# Autodesk Inventor assembly: gameMech_pegged
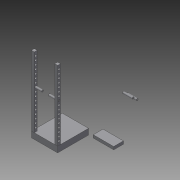
[picture p0: Inventor's stored thumbnail of the model, 180x180]
Saved by Autodesk Inventor 2015 (Build 190159000, 159)
## iProperties
Created: 2015-01-15
Part Number: gameMech_pegged
Document SubType Name: Assembly
Designer: Tucker
Author: Tucker
## Documents named in this file (5)
- C:\Users\Tucker\Documents\GitHub\frc2015\CAD\gameMech_pegged.iam
- C:\Users\Tucker\Documents\GitHub\frc2015\CAD\chasse.ipt
- C:\Users\Tucker\Documents\GitHub\frc2015\CAD\pole.ipt
- C:\Users\Tucker\Documents\GitHub\frc2015\CAD\box_forklift.ipt
- C:\Users\Tucker\Documents\GitHub\frc2015\CAD\axle_word_used_loosely.ipt
## Components (8 placed, 4 different names)
1. chasse:1 — Mate:1, Flush:1, Flush:2, Mate:2, Flush:3, Flush:4
2. pole:1 — Mate:1, Flush:1, Flush:2, Mate:3, Rotation:1, Mate:4
3. pole:2 — Mate:2, Flush:3, Flush:4, Mate:5
4. box_forklift:1
5. axle_word_used_loosely:1 — Mate:3, Rotation:1, Mate:4
6. axle_word_used_loosely:2
7. axle_word_used_loosely:3 — Mate:5
8. axle_word_used_loosely:4
## Relationships (10: Mate 5, Flush 4, RelateRotation 1)
- Mate:1: chasse:1 ↔ pole:1
- Flush:1: chasse:1 ↔ pole:1
- Flush:2: chasse:1 ↔ pole:1
- Mate:2: chasse:1 ↔ pole:2
- Flush:3: chasse:1 ↔ pole:2
- Flush:4: chasse:1 ↔ pole:2
- Mate:3: pole:1 ↔ axle_word_used_loosely:1
- Rotation:1 [RelateRotation] (1 ul): pole:1 ↔ axle_word_used_loosely:1
- Mate:4: pole:1 ↔ axle_word_used_loosely:1
- Mate:5: pole:2 ↔ axle_word_used_loosely:3
